# Autodesk Inventor assembly: battery gate mirrored
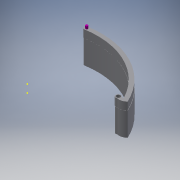
[picture p0: Inventor's stored thumbnail of the model, 180x180]
Saved by Autodesk Inventor 2016 (Build 200138000, 138)
## iProperties
Created: 2015-09-29
Part Number: battery gate mirrored
Document SubType Name: Assembly
Designer: Hulbert Office
Author: Hulbert Office
## Documents named in this file (4)
- C:\Users\Hulbert Office\Dropbox\SHF Robotics\battery gate mirrored.iam
- C:\Users\Hulbert Office\Dropbox\SHF Robotics\battery gate upper mirrored.ipt
- C:\Users\Hulbert Office\Dropbox\SHF Robotics\battery gate mirrored.ipt
- C:\Users\Hulbert Office\Dropbox\SHF Robotics\battery gate pin.ipt
## Components (3 placed, 3 different names)
1. battery gate upper mirrored:1 — Rigid:1, Mate:1
2. battery gate mirrored:1 — Rigid:1
3. battery gate pin:1 — Mate:1
## Relationships (2: WeldJoint 1, Mate 1)
- Rigid:1 [WeldJoint]: battery gate upper mirrored:1 ↔ battery gate mirrored:1
- Mate:1: battery gate upper mirrored:1 ↔ battery gate pin:1
